# Autodesk Inventor assembly: Assembly1
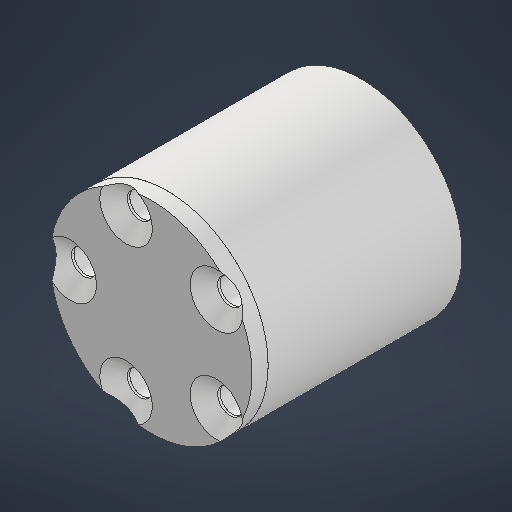
[picture p0: Inventor's stored thumbnail of the model, 512x512]
Saved by Autodesk Inventor 2026.2 (Build 302298010, 298A)
## iProperties
Created: 2026-05-11
Part Number: Assembly1
Document SubType Name: Assembly
Designer: karol
Author: karol
## Documents named in this file (4)
- C:\Users\karol\OneDrive\Dokumenty\GitHub\bolt\bolt\cad\odlew forma\Assembly1.iam
- C:\Users\karol\OneDrive\Dokumenty\GitHub\bolt\bolt\cad\printing parts\rim-v1.ipt
- C:\Users\karol\OneDrive\Dokumenty\GitHub\bolt\bolt\cad\odlew forma\formadol.ipt
- C:\Users\karol\OneDrive\Dokumenty\GitHub\bolt\bolt\cad\odlew forma\forma gora.ipt
## Components (3 placed, 3 different names)
1. rim-v1:1 — Flush:1
2. formadol:1 — Flush:1, Flush:2
3. forma gora:1 — Flush:2
## Relationships (2: Flush 2)
- Flush:1 (0.2032 mm): rim-v1:1 ↔ formadol:1
- Flush:2: formadol:1 ↔ forma gora:1
